# Autodesk Inventor assembly: SM-ZA03
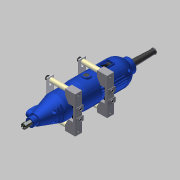
[picture p0: Inventor's stored thumbnail of the model, 180x180]
Saved by Autodesk Inventor 2012 SP1 (Build 160190100, 190)
## iProperties
Created: 2012-04-23
Part Number: SM-ZA03
Document SubType Name: Assembly
Designer: ERF
Mass: 355.059 g
Surface Area: 1046.48 cm^2
Volume: 124.063 cm^3
Density: 2.86192 g/cm^3
Stock Number: SM_ZA03
Author: ERF
Title: Z Axis Spindle Assembly
## Documents named in this file (9)
- C:\Users\eford\Documents\Projects\Shapoko_v1i\Workspaces\Workspace\Projects\USER FOLDER\Edward\Shapeoko_v1i\Assemblies\SM-ZA03.iam
- C:\Users\eford\Documents\Projects\Shapoko_v1i\Workspaces\Workspace\Projects\USER FOLDER\Edward\Shapeoko_v1i\Parts\SM-TM.ipt
- C:\Users\eford\Documents\Projects\Shapoko_v1i\Workspaces\Workspace\Projects\USER FOLDER\Edward\Shapeoko_v1i\Parts\SM-TM3.ipt
- C:\Users\eford\Documents\Projects\Shapoko_v1i\Workspaces\Workspace\Projects\USER FOLDER\Edward\Shapeoko_v1i\Parts\SM-H11.ipt
- C:\Users\eford\Documents\Projects\Shapoko_v1i\Workspaces\Workspace\Projects\USER FOLDER\Edward\Shapeoko_v1i\Parts\SM-H07.ipt
- C:\Users\eford\Documents\Projects\Shapoko_v1i\Workspaces\Workspace\Projects\USER FOLDER\Edward\Shapeoko_v1i\Parts\SM-H03.ipt
- C:\Users\eford\Documents\Projects\Shapoko_v1i\Workspaces\Workspace\Projects\USER FOLDER\Edward\Shapeoko_v1i\Parts\SM-TM2.ipt
- C:\Users\eford\Documents\Projects\Shapoko_v1i\Workspaces\Workspace\Projects\USER FOLDER\Edward\Shapeoko_v1i\Parts\SM-H09.ipt
- C:\Users\eford\Documents\Projects\Shapoko_v1i\Workspaces\Workspace\Projects\USER FOLDER\Edward\Shapeoko_v1i\Parts\SM-H02.ipt
## Components (33 placed, 8 different names)
1. SM-TM:1 — Tangent:1, Flush:6, Insert:13, Insert:14, Flush:7, Flush:8, Mate:18, Insert:17, Mate:20, Insert:27
2. SM-TM3:1 — Tangent:1, Tangent:2, Tangent:3
3. SM-TM:2 — Flush:6, Insert:15, Insert:16, Mate:22, Flush:9, Flush:10, Mate:24, Insert:23, Insert:25
4. SM-H11:1 — Mate:8
5. SM-H11:2 — Mate:11
6. SM-H11:3 — Mate:14
7. SM-H11:4 — Mate:17
8. SM-H07:1 — Insert:9, Mate:14
9. SM-H03:1 — Insert:9, Insert:14
10. SM-H03:2 — Insert:12, Insert:13
11. SM-H03:3 — Insert:10, Insert:15
12. SM-H03:4 — Insert:11, Insert:16
13. SM-H07:2 — Insert:10, Mate:11
14. SM-H07:3 — Insert:11, Mate:17
15. SM-H07:4 — Insert:12, Mate:8
16. SM-TM2:1 — Flush:7, Flush:8, Mate:19, Mate:21, Tangent:2
17. SM-TM2:2 — Flush:9, Flush:10, Mate:23, Mate:25, Tangent:3
18. SM-H09:1 — Insert:22, Mate:22
19. SM-H09:2 — Mate:18, Insert:19
20. SM-H09:3 — Insert:21, Mate:24
21. SM-H09:4 — Insert:20, Mate:20
22. SM-H02:1 — Insert:18
23. SM-H02:2 — Insert:17, Insert:18
24. SM-H03:5 — Insert:19, Mate:19
25. SM-H03:6 — Insert:20, Mate:21
26. SM-H03:7 — Insert:21, Mate:25
27. SM-H03:8 — Insert:22, Mate:23
28. SM-H02:3 — Insert:23, Insert:24
29. SM-H02:4 — Insert:24
30. SM-H02:5 — Insert:25, Insert:26
31. SM-H02:6 — Insert:26
32. SM-H02:7 — Insert:28
33. SM-H02:8 — Insert:27, Insert:28
## Relationships (40: Insert 20, Mate 12, Flush 5, Tangent 3)
- Tangent:1: SM-TM:1 ↔ SM-TM3:1
- Flush:6: SM-TM:1 ↔ SM-TM:2
- Insert:9: SM-H07:1 ↔ SM-H03:1
- Insert:10: SM-H03:3 ↔ SM-H07:2
- Insert:11: SM-H03:4 ↔ SM-H07:3
- Insert:12: SM-H03:2 ↔ SM-H07:4
- Insert:13: SM-TM:1 ↔ SM-H03:2
- Insert:14: SM-TM:1 ↔ SM-H03:1
- Insert:15: SM-TM:2 ↔ SM-H03:3
- Insert:16: SM-TM:2 ↔ SM-H03:4
- Mate:8: SM-H11:1 ↔ SM-H07:4
- Mate:11: SM-H11:2 ↔ SM-H07:2
- Mate:14: SM-H11:3 ↔ SM-H07:1
- Mate:17: SM-H11:4 ↔ SM-H07:3
- Flush:7: SM-TM:1 ↔ SM-TM2:1
- Flush:8: SM-TM:1 ↔ SM-TM2:1
- Mate:18: SM-TM:1 ↔ SM-H09:2
- Insert:17: SM-TM:1 ↔ SM-H02:2
- Insert:18: SM-H02:1 ↔ SM-H02:2
- Insert:19: SM-H09:2 ↔ SM-H03:5
- Mate:19: SM-TM2:1 ↔ SM-H03:5
- Insert:20: SM-H09:4 ↔ SM-H03:6
- Insert:21: SM-H09:3 ↔ SM-H03:7
- Insert:22: SM-H09:1 ↔ SM-H03:8
- Mate:20: SM-TM:1 ↔ SM-H09:4
- Mate:21: SM-TM2:1 ↔ SM-H03:6
- Mate:22: SM-TM:2 ↔ SM-H09:1
- Flush:9: SM-TM:2 ↔ SM-TM2:2
- Flush:10: SM-TM:2 ↔ SM-TM2:2
- Mate:23: SM-TM2:2 ↔ SM-H03:8
- Mate:24: SM-TM:2 ↔ SM-H09:3
- Mate:25: SM-TM2:2 ↔ SM-H03:7
- Insert:23: SM-TM:2 ↔ SM-H02:3
- Tangent:2: SM-TM3:1 ↔ SM-TM2:1
- Tangent:3: SM-TM3:1 ↔ SM-TM2:2
- Insert:24: SM-H02:3 ↔ SM-H02:4
- Insert:25: SM-TM:2 ↔ SM-H02:5
- Insert:26: SM-H02:5 ↔ SM-H02:6
- Insert:27: SM-TM:1 ↔ SM-H02:8
- Insert:28: SM-H02:7 ↔ SM-H02:8
